# Autodesk Inventor assembly: Senior Project Assembly
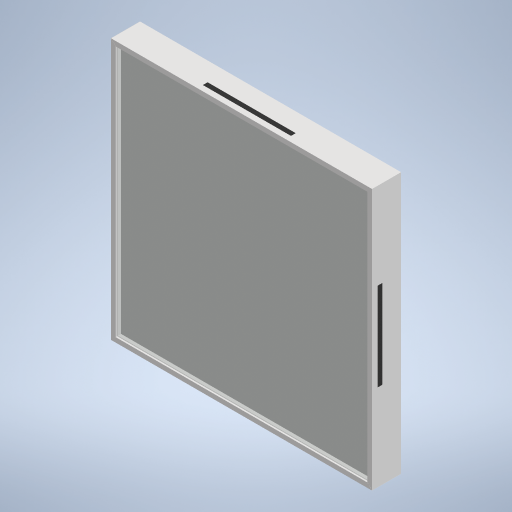
[picture p0: Inventor's stored thumbnail of the model, 512x512]
Saved by Autodesk Inventor 2024.2 (Build 282272000, 272)
## iProperties
Created: 2024-02-22
Part Number: Senior Project Assembly
Document SubType Name: Assembly
Designer: flynf
Author: flynf
## Documents named in this file (4)
- C:\Users\flynf\Documents\Senior Project Assembly.iam
- C:\Users\flynf\Documents\Final Product backplate.ipt
- C:\Users\flynf\Documents\Frame Side(Short).ipt
- C:\Users\flynf\Documents\Clear Panel.ipt
## Components (6 placed, 3 different names)
1. Final Product backplate:1 — Flush:3, Mate:8, Mate:9, Mate:10, Mate:11, Flush:4, Mate:14, Mate:15, Mate:16, Mate:17
2. Clear Panel:1 — Mate:12, Mate:13
3. Frame Side(Short):2 — Flush:3, Mate:8, Mate:9, Mate:13
4. Frame Side(Short):3 — Mate:10, Mate:11, Flush:4, Mate:12, Flush:5
5. Frame Side(Short):4 — Flush:5, Mate:14, Mate:15, Flush:6
6. Frame Side(Short):5 — Flush:6, Mate:16, Mate:17
## Relationships (14: Mate 10, Flush 4)
- Flush:3: Final Product backplate:1 ↔ Frame Side(Short):2
- Mate:8: Final Product backplate:1 ↔ Frame Side(Short):2
- Mate:9: Final Product backplate:1 ↔ Frame Side(Short):2
- Mate:10: Final Product backplate:1 ↔ Frame Side(Short):3
- Mate:11: Final Product backplate:1 ↔ Frame Side(Short):3
- Flush:4: Final Product backplate:1 ↔ Frame Side(Short):3
- Mate:12: Clear Panel:1 ↔ Frame Side(Short):3
- Mate:13: Clear Panel:1 ↔ Frame Side(Short):2
- Flush:5: Frame Side(Short):3 ↔ Frame Side(Short):4
- Mate:14: Final Product backplate:1 ↔ Frame Side(Short):4
- Mate:15: Final Product backplate:1 ↔ Frame Side(Short):4
- Flush:6: Frame Side(Short):4 ↔ Frame Side(Short):5
- Mate:16: Final Product backplate:1 ↔ Frame Side(Short):5
- Mate:17: Final Product backplate:1 ↔ Frame Side(Short):5
